# Autodesk Inventor assembly: fullSparFlat
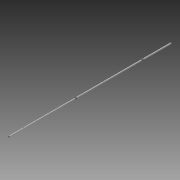
[picture p0: Inventor's stored thumbnail of the model, 180x180]
Saved by Autodesk Inventor 2014 (Build 180170000, 170)
## iProperties
Created: 2015-03-27
Part Number: fullSparFlat
Document SubType Name: Assembly
Designer: ddeboer
Author: ddeboer
## Documents named in this file (4)
- C:\Users\ddeboer\Desktop\hera-cad\surface\sparFullFlat_US.iam
- C:\Users\ddeboer\Desktop\hera-cad\surface\pvcSection_2in.ipt
- C:\Users\ddeboer\Desktop\hera-cad\smallParts\coupler_2in.ipt
- C:\Users\ddeboer\Desktop\hera-cad\surface\pvcSection_2in_cut4full.ipt
## Components (5 placed, 3 different names)
1. pvcSection_2in:2 — Insert:2, Insert:3
2. coupler_2in:1 — Insert:3, Insert:4
3. coupler_2in:2 — Insert:2, Insert:5
4. pvcSection_2in_cut4full:1 — Insert:4
5. pvcSection_2in:3 — Insert:5
## Relationships (4: Insert 4)
- Insert:2 (-29.3624 mm): pvcSection_2in:2 ↔ coupler_2in:2
- Insert:3 (-29.3624 mm): pvcSection_2in:2 ↔ coupler_2in:1
- Insert:4 (-29.3624 mm): coupler_2in:1 ↔ pvcSection_2in_cut4full:1
- Insert:5 (-29.3624 mm): coupler_2in:2 ↔ pvcSection_2in:3
